# Autodesk Inventor assembly: mill_assembly
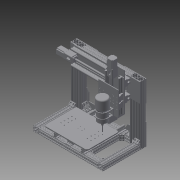
[picture p0: Inventor's stored thumbnail of the model, 180x180]
Saved by Autodesk Inventor 2014 (Build 180170000, 170)
## iProperties
Created: 2014-08-08
Part Number: mill_assembly
Document SubType Name: Assembly
Designer: Matthew
Author: Matthew
## Documents named in this file (45)
- C:\Users\Matthew\Documents\GitHub\CNC Mill\mill_assembly.iam
- C:\Users\Matthew\Documents\GitHub\CNC Mill\8020\2020.ipt
- C:\Users\Matthew\Documents\GitHub\CNC Mill\8020\2020_18in.ipt
- C:\Users\Matthew\Documents\GitHub\CNC Mill\8020\gusset_4138.ipt
- C:\Users\Matthew\Documents\GitHub\CNC Mill\8020\gusset_4134.ipt
- C:\Users\Matthew\Documents\GitHub\CNC Mill\mic6_plate.ipt
- C:\Users\Matthew\Documents\GitHub\CNC Mill\1605\1605_400mm.ipt
- C:\Users\Matthew\Documents\GitHub\CNC Mill\1605\1605_ballnut.ipt
- C:\Users\Matthew\Documents\GitHub\CNC Mill\nema23_motor_mount.ipt
- C:\Users\Matthew\Documents\GitHub\CNC Mill\6.35x10mm_coupler.ipt
- C:\Users\Matthew\Documents\GitHub\CNC Mill\sbr\sbr20\sbr20_400mm.ipt
- C:\Users\Matthew\Documents\GitHub\CNC Mill\HD16.ipt
- C:\Users\Matthew\Documents\GitHub\CNC Mill\nema23_HS8630.ipt
- C:\Users\Matthew\Documents\GitHub\CNC Mill\z-axis_mount_plate.ipt
- C:\Users\Matthew\Documents\GitHub\CNC Mill\y-axis_mount_plate.ipt
- C:\Users\Matthew\Documents\GitHub\CNC Mill\router_plate.ipt
- C:\Users\Matthew\Documents\GitHub\CNC Mill\router_mount.ipt
- C:\Users\Matthew\Documents\GitHub\CNC Mill\1617evs.ipt
- C:\Users\Matthew\Documents\GitHub\CNC Mill\ff12_mount.ipt
- C:\Users\Matthew\Documents\GitHub\CNC Mill\ff12.ipt
- C:\Users\Matthew\Documents\GitHub\CNC Mill\sbr\sbr20\sbr20_500mm.ipt
- C:\Users\Matthew\Documents\GitHub\CNC Mill\1605\1605_500mm.ipt
- C:\Users\Matthew\Documents\GitHub\CNC Mill\sbr\sbr20\sbr20_300mm.ipt
- C:\Users\Matthew\Documents\GitHub\CNC Mill\8020\2040_top_bar.ipt
- C:\Users\Matthew\Documents\GitHub\CNC Mill\8020\2040_uprights.ipt
- C:\Users\Matthew\Downloads\Imported Components\endmill 2 flute_finishing\endmill 2 flute_finishing.ipt
- C:\Users\Matthew\Downloads\Imported Components\User Library-ER COLLET\Assembly1.iam
- C:\Users\Matthew\Documents\GitHub\CNC Mill\8020\2020_rear.ipt
- C:\Users\Matthew\Documents\GitHub\CNC Mill\8020\2020_front.ipt
- C:\Users\Matthew\Documents\GitHub\CNC Mill\1605\1605_300mm.ipt
- C:\Users\Matthew\Documents\GitHub\CNC Mill\hd16_standoff.ipt
- C:\Users\Matthew\Documents\GitHub\CNC Mill\sbr20uu_standoff.ipt
- C:\Users\Matthew\Documents\GitHub\CNC Mill\versaframe\versaframe_30in.ipt
- C:\Users\Matthew\Documents\GitHub\CNC Mill\versaframe\versaframe_35in.ipt
- C:\Users\Matthew\Documents\GitHub\CNC Mill\versaframe\versaframe_7.5n.ipt
- C:\Users\Matthew\Documents\GitHub\CNC Mill\8020\2040-2040_left.iam
- C:\Users\Matthew\Documents\GitHub\CNC Mill\8020\2040-2040_right.iam
- C:\Users\Matthew\Documents\GitHub\CNC Mill\8020\2020-2040_right.iam
- C:\Users\Matthew\Documents\GitHub\CNC Mill\8020\2020-2040_left.iam
- C:\Users\Matthew\Documents\GitHub\CNC Mill\fk12.ipt
- C:\Users\Matthew\Documents\GitHub\CNC Mill\sbr\sbr20\sbr20uu.ipt
- C:\Users\Matthew\Documents\GitHub\CNC Mill\m6x1.ipt
- C:\Users\Matthew\Documents\GitHub\CNC Mill\m5x0.8.ipt
- C:\Users\Matthew\Documents\GitHub\CNC Mill\8020\SHCS bolt.ipt
- C:\Users\Matthew\Documents\GitHub\CNC Mill\8020\0.5in_tnut.iam
## Components (155 placed, 44 different names)
1. 2020_18in:1 — Mate:31, Mate:32, Mate:38, Mate:47, Mate:48, Flush:161, Flush:168, Mate:253
2. 2020_18in:2 — Mate:28, Mate:29, Mate:34, Mate:241, Flush:163, Mate:242, Flush:164, Mate:255, Flush:171, Flush:172, Mate:394
3. gusset_4138:1 — Mate:260, Mate:261, Flush:175
4. gusset_4138:2 — Mate:258, Mate:259, Mate:262, Flush:175
5. gusset_4134:1 — Mate:28, Mate:29, Mate:275
6. gusset_4134:2 — Mate:31, Mate:32, Mate:276, Insert:58, Insert:60, Insert:61, Insert:62
7. gusset_4134:3 — Mate:34, Flush:61, Flush:147, Mate:278
8. gusset_4134:4 — Mate:38, Flush:62, Flush:153, Mate:279
9. gusset_4134:6 — Mate:47, Mate:48, Flush:61, Flush:62, Mate:269, Flush:401, Flush:402, Flush:403
10. mic6_plate:1 — Mate:293, Flush:352, Insert:17, Insert:18, Insert:19, Insert:20, Insert:21, Insert:22, Insert:23, Insert:24, Insert:25, Insert:26, Insert:27, Insert:28, Insert:29, Insert:30, Insert:31, Insert:32, Insert:33, Insert:34, Insert:35, Insert:36, Flush:395
11. 1605_400mm:1 — Mate:108, Insert:2, Insert:13, Insert:16
12. 1605_ballnut:1 — Mate:108, Mate:133, Mate:134, Flush:75
13. nema23_motor_mount:1 — Mate:136, Mate:254, Flush:192, Flush:193, Mate:317, Flush:329, Flush:330
14. nema23_motor_mount:2 — Mate:154, Flush:321, Flush:322, Mate:316, Flush:327, Flush:328, Mate:364, Flush:376
15. 1605_ballnut:6 — Mate:158, Flush:90, Mate:159, Mate:282
16. 6.35x10mm_coupler:1 — Insert:4, Insert:14
17. sbr20_400mm:1 — Flush:136, Mate:247, Flush:191, Mate:318
18. sbr20_400mm:2 — Flush:136, Mate:248, Flush:190, Mate:328
19. HD16:1 — Mate:133, Mate:134, Flush:75, Flush:194, Mate:283, Mate:284, Mate:326, Mate:329, Flush:352, Mate:339
20. nema23_HS8630:1 — Mate:136, Flush:192, Flush:193
21. 6.35x10mm_coupler:2 — Insert:2
22. z-axis_mount_plate:1 — Mate:361, Flush:370, Flush:371, Flush:372, Flush:373, Mate:362, Mate:363, Flush:375, Mate:364, Flush:376, Flush:390, Flush:392
23. nema23_HS8630:2 — Mate:154, Insert:4, Flush:321, Flush:322
24. HD16:6 — Mate:158, Flush:90, Mate:159, Mate:186, Flush:120, Flush:121, Mate:210, Mate:211, Mate:378, Mate:379, Flush:389, Flush:390
25. y-axis_mount_plate:1 — Mate:177, Mate:199, Mate:200, Flush:135, Mate:206, Flush:137, Flush:184, Mate:267, Flush:396
26. nema23_motor_mount:4 — Mate:177, Flush:137, Flush:323, Flush:324, Mate:315, Flush:325, Flush:326
27. 6.35x10mm_coupler:3
28. nema23_HS8630:3 — Flush:323, Flush:324
29. 1605_ballnut:7 — Mate:240
30. HD16:7 — Mate:203, Mate:205, Mate:348, Mate:351, Mate:352, Flush:364
31. router_plate:1 — Mate:186, Flush:120, Flush:121, Mate:187, Flush:122, Flush:123, Mate:381, Flush:391, Flush:392, Mate:383, Flush:393, Flush:394, Insert:37, Insert:38, Insert:39, Insert:40, Insert:41, Insert:42, Insert:43, Insert:44, Insert:45, Insert:46, Insert:47, Insert:48, Insert:49, Insert:50, Insert:51, Insert:52, Insert:53, Insert:54, Insert:55, Insert:56
32. router_mount:1 — Insert:7, Mate:187, Flush:122, Flush:123, Mate:383, Flush:393, Flush:394
33. 1617evs:1 — Insert:7
34. ff12_mount:1 — Insert:9, Mate:256, Flush:331
35. ff12:1 — Insert:9, Insert:13
36. sbr20_500mm:1 — Flush:133, Mate:200, Mate:203, Flush:135, Mate:346, Flush:371, Mate:382
37. sbr20_500mm:2 — Flush:133, Mate:199, Mate:205, Mate:347
38. 1605_500mm:1 — Insert:11, Mate:240, Insert:15
39. ff12:2 — Insert:11, Insert:12
40. ff12_mount:2 — Insert:12, Mate:206
41. sbr20_300mm:1 — Flush:138, Mate:210, Flush:372, Mate:363, Flush:374, Flush:375, Mate:371
42. sbr20_300mm:2 — Flush:138, Mate:211, Flush:373, Mate:362, Flush:374, Mate:377
43. 2020:1 — Mate:223, Mate:230, Mate:233, Mate:248, Mate:250, Flush:169, Flush:190, Mate:389
44. 2020:2 — Mate:222, Mate:224, Mate:226, Mate:247, Mate:251, Flush:170, Flush:191, Mate:391
45. gusset_4134:8 — Mate:222, Flush:147, Mate:277
46. gusset_4134:9 — Mate:223, Flush:149, Flush:150, Flush:151, Mate:280, Flush:401
47. gusset_4134:11 — Mate:224, Flush:149, Mate:268
48. gusset_4134:12 — Mate:230, Flush:151, Mate:390
49. gusset_4134:13 — Mate:226, Flush:150, Mate:281
50. gusset_4134:14 — Flush:153, Mate:233
51. 2040_top_bar:1 — Mate:257, Flush:173, Flush:174, Mate:258, Mate:261, Flush:184, Mate:267, Flush:313, Flush:315
52. 2040_uprights:1 — Flush:161, Mate:241, Flush:167, Mate:252, Flush:168, Mate:253, Mate:257, Flush:173, Flush:174, Mate:259, Mate:262, Mate:269, Mate:276, Mate:311, Flush:314, Mate:314, Flush:319, Flush:320, Flush:396, Flush:398, Mate:385, Flush:400
53. endmill 2 flute_finishing:1
54. Assembly1:1 [sub-assembly]
55. 2040_uprights:2 — Flush:163, Mate:242, Flush:164, Mate:249, Flush:165, Flush:166, Mate:260, Mate:275, Flush:208, Mate:312, Flush:316, Mate:313, Flush:317, Flush:318, Mate:339, Mate:386, Flush:399, Flush:404, Mate:393
56. 2020_rear:1 — Mate:249, Flush:165, Flush:166, Mate:250, Mate:251, Flush:167, Mate:252, Flush:169, Flush:170, Mate:254, Mate:268, Mate:280, Flush:221, Mate:384, Mate:387, Mate:388, Mate:392
57. 2020_front:1 — Mate:255, Flush:171, Flush:172, Mate:256, Mate:277, Mate:278, Mate:279, Mate:281, Flush:331, Mate:390
58. 1605_300mm:1 — Insert:14, Mate:282
59. hd16_standoff:1 — Flush:194, Mate:283, Mate:284, Mate:293
60. versaframe_30in:1 — Flush:200, Flush:201, Mate:294, Flush:202, Flush:203, Mate:295, Flush:205, Flush:206, Flush:228, Flush:230
61. versaframe_30in:2 — Flush:200, Flush:201, Flush:204, Flush:221
62. versaframe_35in:1 — Mate:294, Flush:202, Flush:203, Flush:204, Flush:208, Flush:213, Mate:303, Flush:229
63. versaframe_35in:2 — Mate:295, Flush:205, Flush:206, Mate:297, Flush:209, Flush:210, Mate:304, Flush:231
64. versaframe_30in:3 — Mate:297, Flush:209, Flush:210, Flush:211, Flush:212, Flush:232, Flush:233, Mate:305
65. versaframe_30in:4 — Flush:211, Flush:212, Flush:213, Flush:220, Flush:308, Flush:235, Flush:309
66. versaframe_7.5n:1 — Flush:308, Flush:235, Flush:309, Flush:310, Flush:311, Mate:307, Mate:308
67. versaframe_7.5n:2 — Flush:232, Flush:233, Mate:305, Mate:306, Flush:234, Mate:309, Mate:310, Flush:312
68. versaframe_30in:5 — Flush:220, Flush:222, Mate:306, Flush:234, Flush:310
69. versaframe_30in:6 — Flush:222, Flush:311, Mate:307, Mate:308
70. versaframe_7.5n:3 — Mate:303, Flush:228, Flush:229
71. versaframe_7.5n:4 — Mate:304, Flush:230, Flush:231
72. versaframe_30in:7
73. versaframe_30in:8 — Mate:309, Mate:310, Flush:312
74. 2040-2040_left:1 [sub-assembly] — Mate:311, Flush:313, Flush:314
75. 2040-2040_right:1 [sub-assembly] — Mate:312, Flush:315, Flush:316
76. 2020-2040_right:1 [sub-assembly] — Mate:313, Flush:317, Flush:318
77. 2020-2040_left:1 [sub-assembly] — Mate:314, Flush:319, Flush:320
78. fk12:1 — Insert:15, Mate:315, Flush:325, Flush:326, Mate:382
79. fk12:2 — Mate:316, Flush:327, Flush:328
80. fk12:3 — Mate:317, Flush:329, Flush:330, Insert:16
81. sbr20uu:1 — Flush:332, Mate:319, Flush:333, Mate:332, Flush:347, Mate:333
82. sbr20uu:2 — Mate:318, Flush:332, Mate:319, Flush:333, Mate:326, Mate:335, Flush:349, Mate:336, Flush:395
83. sbr20uu:3 — Flush:344, Mate:327, Flush:345, Mate:328, Mate:329, Flush:350, Mate:337, Mate:338
84. sbr20uu:13 — Flush:344, Mate:327, Flush:345, Mate:330, Flush:346, Mate:331
85. sbr20uu_standoff:4 — Mate:330, Flush:346, Mate:331
86. sbr20uu_standoff:5 — Mate:332, Flush:347, Mate:333
87. sbr20uu_standoff:6 — Mate:335, Flush:349, Mate:336, Flush:353
88. sbr20uu_standoff:7 — Flush:350, Mate:337, Mate:338, Flush:353
89. m6x1:1 — Insert:24
90. m6x1:2 — Insert:21
91. m6x1:3 — Insert:17
92. m6x1:4 — Insert:20
93. m6x1:5 — Insert:18
94. m6x1:6 — Insert:19
95. m6x1:7 — Insert:22
96. m6x1:8 — Insert:23
97. m6x1:9 — Insert:28
98. m6x1:10 — Insert:27
99. m6x1:11 — Insert:32
100. m6x1:12 — Insert:26
101. m6x1:13 — Insert:29
102. m6x1:14 — Insert:30
103. m6x1:15 — Insert:25
104. m6x1:16 — Insert:31
105. m5x0.8:1 — Insert:36
106. m5x0.8:2 — Insert:34
107. m5x0.8:3 — Insert:33
108. m5x0.8:4 — Insert:35
109. sbr20uu:14 — Mate:347, Flush:362, Mate:348, Mate:355, Flush:366, Mate:356, Flush:370
110. sbr20uu:15 — Mate:353, Mate:354, Flush:365
111. sbr20uu:18 — Mate:346, Flush:362, Mate:358, Mate:359, Flush:368
112. sbr20uu:19 — Mate:357, Flush:367, Mate:360
113. sbr20uu_standoff:8 — Mate:353, Mate:354, Flush:365, Flush:369
114. hd16_standoff:2 — Mate:351, Mate:352, Flush:364, Mate:361
115. sbr20uu_standoff:9 — Mate:355, Flush:366, Mate:356
116. sbr20uu_standoff:10 — Mate:358, Mate:359, Flush:368
117. sbr20uu_standoff:11 — Mate:357, Flush:367, Mate:360, Flush:369
118. sbr20uu:22 — Mate:371
119. sbr20uu:23 — Flush:387, Flush:391
120. sbr20uu_standoff:12
121. sbr20uu_standoff:13 — Flush:388
122. sbr20uu:24
123. sbr20uu:25 — Mate:377, Flush:387, Mate:380
124. sbr20uu_standoff:14
125. sbr20uu_standoff:15 — Flush:388
126. hd16_standoff:3 — Mate:378, Mate:379, Flush:389, Mate:380, Mate:381
127. m6x1:18 — Insert:48
128. m6x1:19 — Insert:40
129. m6x1:20 — Insert:42
130. m6x1:21 — Insert:50
131. m6x1:22 — Insert:51
132. m6x1:23 — Insert:47
133. m6x1:24 — Insert:52
134. m6x1:25 — Insert:39
135. m6x1:26 — Insert:41
136. m6x1:27 — Insert:49
137. m6x1:28 — Insert:38
138. m6x1:29 — Insert:44
139. m6x1:30 — Insert:43
140. m6x1:31 — Insert:46
141. m6x1:32 — Insert:37
142. m6x1:33 — Insert:45
143. m5x0.8:5 — Insert:53
144. m5x0.8:6 — Insert:54
145. m5x0.8:7 — Insert:55
146. m5x0.8:8 — Insert:56
147. gusset_4138:5 — Mate:384, Flush:398, Mate:385
148. gusset_4138:6 — Mate:386, Flush:399, Mate:387
149. gusset_4134:15 — Mate:388, Mate:389, Flush:400, Flush:402
150. gusset_4134:16 — Mate:391, Flush:403, Flush:404, Mate:392, Flush:405
151. gusset_4134:17 — Mate:393, Mate:394, Flush:405
152. SHCS bolt:2 — Insert:58
153. 0.5in_tnut:2 [sub-assembly] — Insert:60
154. 0.5in_tnut:3 [sub-assembly] — Insert:61
155. SHCS bolt:3 — Insert:62
## Relationships (344: Mate 148, Flush 141, Insert 55)
- Mate:28: 2020_18in:2 ↔ gusset_4134:1
- Mate:29: 2020_18in:2 ↔ gusset_4134:1
- Mate:31: 2020_18in:1 ↔ gusset_4134:2
- Mate:32: 2020_18in:1 ↔ gusset_4134:2
- Mate:34: 2020_18in:2 ↔ gusset_4134:3
- Mate:38: 2020_18in:1 ↔ gusset_4134:4
- Mate:47: 2020_18in:1 ↔ gusset_4134:6
- Mate:48: 2020_18in:1 ↔ gusset_4134:6
- Mate:108: 1605_400mm:1 ↔ 1605_ballnut:1
- Flush:61: gusset_4134:3 ↔ gusset_4134:6
- Flush:62: gusset_4134:4 ↔ gusset_4134:6
- Mate:133: 1605_ballnut:1 ↔ HD16:1
- Mate:134: 1605_ballnut:1 ↔ HD16:1
- Flush:75: 1605_ballnut:1 ↔ HD16:1
- Insert:2 (-12.5 mm): 1605_400mm:1 ↔ 6.35x10mm_coupler:2
- Mate:136: nema23_motor_mount:1 ↔ nema23_HS8630:1
- Mate:154: nema23_motor_mount:2 ↔ nema23_HS8630:2
- Insert:4 (-7 mm): 6.35x10mm_coupler:1 ↔ nema23_HS8630:2
- Mate:158: 1605_ballnut:6 ↔ HD16:6
- Flush:90: 1605_ballnut:6 ↔ HD16:6
- Mate:159: 1605_ballnut:6 ↔ HD16:6
- [Mate]: nema23_motor_mount:4 ↔ nema23_HS8630:3
- [Insert] (-7 mm): 6.35x10mm_coupler:3 ↔ nema23_HS8630:3
- [Mate]: 1605_ballnut:7 ↔ HD16:7
- [Flush]: 1605_ballnut:7 ↔ HD16:7
- [Mate]: 1605_ballnut:7 ↔ HD16:7
- Mate:177: y-axis_mount_plate:1 ↔ nema23_motor_mount:4
- Insert:7: router_mount:1 ↔ 1617evs:1
- Mate:186: HD16:6 ↔ router_plate:1
- Flush:120 (-96.7994 mm): HD16:6 ↔ router_plate:1
- Flush:121 (64.897 mm): HD16:6 ↔ router_plate:1
- Mate:187: router_plate:1 ↔ router_mount:1
- Flush:122: router_plate:1 ↔ router_mount:1
- Flush:123 (44.45 mm): router_plate:1 ↔ router_mount:1
- Insert:9: ff12_mount:1 ↔ ff12:1
- Flush:133: sbr20_500mm:1 ↔ sbr20_500mm:2
- Mate:199: y-axis_mount_plate:1 ↔ sbr20_500mm:2
- Mate:200: y-axis_mount_plate:1 ↔ sbr20_500mm:1
- Mate:203 (19.9 mm): HD16:7 ↔ sbr20_500mm:1
- Mate:205 (19.9 mm): HD16:7 ↔ sbr20_500mm:2
- Flush:135: y-axis_mount_plate:1 ↔ sbr20_500mm:1
- Flush:136: sbr20_400mm:1 ↔ sbr20_400mm:2
- Insert:11: 1605_500mm:1 ↔ ff12:2
- Insert:12: ff12:2 ↔ ff12_mount:2
- Mate:206: y-axis_mount_plate:1 ↔ ff12_mount:2
- Insert:13: 1605_400mm:1 ↔ ff12:1
- Flush:137: y-axis_mount_plate:1 ↔ nema23_motor_mount:4
- Flush:138: sbr20_300mm:1 ↔ sbr20_300mm:2
- Mate:210 (11 mm): HD16:6 ↔ sbr20_300mm:1
- Mate:211 (11 mm): HD16:6 ↔ sbr20_300mm:2
- Mate:222: 2020:2 ↔ gusset_4134:8
- Flush:147: gusset_4134:3 ↔ gusset_4134:8
- Mate:223: 2020:1 ↔ gusset_4134:9
- Mate:224: 2020:2 ↔ gusset_4134:11
- Mate:226: 2020:2 ↔ gusset_4134:13
- Flush:149: gusset_4134:9 ↔ gusset_4134:11
- Mate:230: 2020:1 ↔ gusset_4134:12
- Flush:150: gusset_4134:9 ↔ gusset_4134:13
- Flush:151: gusset_4134:9 ↔ gusset_4134:12
- Flush:153: gusset_4134:4 ↔ gusset_4134:14
- Mate:233: 2020:1 ↔ gusset_4134:14
- Mate:240: 1605_ballnut:7 ↔ 1605_500mm:1
- Flush:161: 2020_18in:1 ↔ 2040_uprights:1
- Mate:241: 2020_18in:2 ↔ 2040_uprights:1
- Flush:163: 2020_18in:2 ↔ 2040_uprights:2
- Mate:242: 2020_18in:2 ↔ 2040_uprights:2
- Flush:164: 2020_18in:2 ↔ 2040_uprights:2
- Mate:247: sbr20_400mm:1 ↔ 2020:2
- Mate:248: sbr20_400mm:2 ↔ 2020:1
- Mate:249: 2040_uprights:2 ↔ 2020_rear:1
- Flush:165: 2040_uprights:2 ↔ 2020_rear:1
- Flush:166: 2040_uprights:2 ↔ 2020_rear:1
- Mate:250: 2020:1 ↔ 2020_rear:1
- Mate:251: 2020:2 ↔ 2020_rear:1
- Flush:167: 2040_uprights:1 ↔ 2020_rear:1
- Mate:252: 2040_uprights:1 ↔ 2020_rear:1
- Flush:168: 2020_18in:1 ↔ 2040_uprights:1
- Mate:253: 2020_18in:1 ↔ 2040_uprights:1
- Flush:169: 2020:1 ↔ 2020_rear:1
- Flush:170: 2020:2 ↔ 2020_rear:1
- Mate:254: nema23_motor_mount:1 ↔ 2020_rear:1
- Mate:255: 2020_18in:2 ↔ 2020_front:1
- Flush:171: 2020_18in:2 ↔ 2020_front:1
- Flush:172: 2020_18in:2 ↔ 2020_front:1
- Mate:256: ff12_mount:1 ↔ 2020_front:1
- Mate:257: 2040_top_bar:1 ↔ 2040_uprights:1
- Flush:173: 2040_top_bar:1 ↔ 2040_uprights:1
- Flush:174: 2040_top_bar:1 ↔ 2040_uprights:1
- Mate:258: gusset_4138:2 ↔ 2040_top_bar:1
- Mate:259: gusset_4138:2 ↔ 2040_uprights:1
- Mate:260: gusset_4138:1 ↔ 2040_uprights:2
- Mate:261: gusset_4138:1 ↔ 2040_top_bar:1
- Mate:262: gusset_4138:2 ↔ 2040_uprights:1
- Flush:175: gusset_4138:1 ↔ gusset_4138:2
- Flush:184: y-axis_mount_plate:1 ↔ 2040_top_bar:1
- Mate:267: y-axis_mount_plate:1 ↔ 2040_top_bar:1
- Mate:268: gusset_4134:11 ↔ 2020_rear:1
- Mate:269: gusset_4134:6 ↔ 2040_uprights:1
- Flush:190: sbr20_400mm:2 ↔ 2020:1
- Flush:191: sbr20_400mm:1 ↔ 2020:2
- Mate:275: gusset_4134:1 ↔ 2040_uprights:2
- Mate:276: gusset_4134:2 ↔ 2040_uprights:1
- Mate:277: gusset_4134:8 ↔ 2020_front:1
- Mate:278: gusset_4134:3 ↔ 2020_front:1
- Mate:279: gusset_4134:4 ↔ 2020_front:1
- Mate:280: gusset_4134:9 ↔ 2020_rear:1
- Mate:281: gusset_4134:13 ↔ 2020_front:1
- Insert:14 (-12.5 mm): 6.35x10mm_coupler:1 ↔ 1605_300mm:1
- Mate:282: 1605_ballnut:6 ↔ 1605_300mm:1
- Flush:192 (-0.889 mm): nema23_motor_mount:1 ↔ nema23_HS8630:1
- Flush:193: nema23_motor_mount:1 ↔ nema23_HS8630:1
- Flush:194: HD16:1 ↔ hd16_standoff:1
- Mate:283: HD16:1 ↔ hd16_standoff:1
- Mate:284: HD16:1 ↔ hd16_standoff:1
- Mate:293: mic6_plate:1 ↔ hd16_standoff:1
- Flush:200: versaframe_30in:1 ↔ versaframe_30in:2
- Flush:201: versaframe_30in:1 ↔ versaframe_30in:2
- Mate:294: versaframe_30in:1 ↔ versaframe_35in:1
- Flush:202: versaframe_30in:1 ↔ versaframe_35in:1
- Flush:203: versaframe_30in:1 ↔ versaframe_35in:1
- Flush:204: versaframe_30in:2 ↔ versaframe_35in:1
- Mate:295: versaframe_30in:1 ↔ versaframe_35in:2
- Flush:205: versaframe_30in:1 ↔ versaframe_35in:2
- Flush:206: versaframe_30in:1 ↔ versaframe_35in:2
- Flush:208: 2040_uprights:2 ↔ versaframe_35in:1
- Mate:297: versaframe_35in:2 ↔ versaframe_30in:3
- Flush:209: versaframe_35in:2 ↔ versaframe_30in:3
- Flush:210: versaframe_35in:2 ↔ versaframe_30in:3
- Flush:211: versaframe_30in:3 ↔ versaframe_30in:4
- Flush:212: versaframe_30in:3 ↔ versaframe_30in:4
- Flush:213: versaframe_35in:1 ↔ versaframe_30in:4
- Flush:220: versaframe_30in:4 ↔ versaframe_30in:5
- Flush:221: 2020_rear:1 ↔ versaframe_30in:2
- Flush:222: versaframe_30in:5 ↔ versaframe_30in:6
- Mate:303: versaframe_35in:1 ↔ versaframe_7.5n:3
- Flush:228: versaframe_30in:1 ↔ versaframe_7.5n:3
- Flush:229: versaframe_35in:1 ↔ versaframe_7.5n:3
- Mate:304: versaframe_35in:2 ↔ versaframe_7.5n:4
- Flush:230: versaframe_30in:1 ↔ versaframe_7.5n:4
- Flush:231: versaframe_35in:2 ↔ versaframe_7.5n:4
- Flush:232: versaframe_30in:3 ↔ versaframe_7.5n:2
- Flush:233: versaframe_30in:3 ↔ versaframe_7.5n:2
- Mate:305: versaframe_30in:3 ↔ versaframe_7.5n:2
- Mate:306: versaframe_7.5n:2 ↔ versaframe_30in:5
- Flush:234: versaframe_7.5n:2 ↔ versaframe_30in:5
- Flush:308: versaframe_30in:4 ↔ versaframe_7.5n:1
- Flush:235: versaframe_30in:4 ↔ versaframe_7.5n:1
- Flush:309: versaframe_30in:4 ↔ versaframe_7.5n:1
- Flush:310: versaframe_7.5n:1 ↔ versaframe_30in:5
- Flush:311: versaframe_7.5n:1 ↔ versaframe_30in:6
- Mate:307: versaframe_7.5n:1 ↔ versaframe_30in:6
- Mate:308: versaframe_7.5n:1 ↔ versaframe_30in:6
- Mate:309: versaframe_7.5n:2 ↔ versaframe_30in:8
- Mate:310: versaframe_7.5n:2 ↔ versaframe_30in:8
- Flush:312: versaframe_7.5n:2 ↔ versaframe_30in:8
- Mate:311: 2040_uprights:1 ↔ 2040-2040_left:1
- Flush:313: 2040_top_bar:1 ↔ 2040-2040_left:1
- Flush:314: 2040_uprights:1 ↔ 2040-2040_left:1
- Mate:312: 2040_uprights:2 ↔ 2040-2040_right:1
- Flush:315: 2040_top_bar:1 ↔ 2040-2040_right:1
- Flush:316: 2040_uprights:2 ↔ 2040-2040_right:1
- Mate:313: 2040_uprights:2 ↔ 2020-2040_right:1
- Flush:317: 2040_uprights:2 ↔ 2020-2040_right:1
- Flush:318: 2040_uprights:2 ↔ 2020-2040_right:1
- Mate:314: 2040_uprights:1 ↔ 2020-2040_left:1
- Flush:319: 2040_uprights:1 ↔ 2020-2040_left:1
- Flush:320: 2040_uprights:1 ↔ 2020-2040_left:1
- Flush:321 (-0.889 mm): nema23_motor_mount:2 ↔ nema23_HS8630:2
- Flush:322 (0.889 mm): nema23_motor_mount:2 ↔ nema23_HS8630:2
- Flush:323 (-0.889 mm): nema23_motor_mount:4 ↔ nema23_HS8630:3
- Flush:324: nema23_motor_mount:4 ↔ nema23_HS8630:3
- Insert:15: 1605_500mm:1 ↔ fk12:1
- Mate:315: nema23_motor_mount:4 ↔ fk12:1
- Flush:325 (6.1305 mm): nema23_motor_mount:4 ↔ fk12:1
- Flush:326 (6.1305 mm): nema23_motor_mount:4 ↔ fk12:1
- Mate:316: nema23_motor_mount:2 ↔ fk12:2
- Flush:327 (-6.1305 mm): nema23_motor_mount:2 ↔ fk12:2
- Flush:328 (6.1305 mm): nema23_motor_mount:2 ↔ fk12:2
- Mate:317: nema23_motor_mount:1 ↔ fk12:3
- Flush:329 (6.1305 mm): nema23_motor_mount:1 ↔ fk12:3
- Flush:330 (6.1305 mm): nema23_motor_mount:1 ↔ fk12:3
- Insert:16: 1605_400mm:1 ↔ fk12:3
- Flush:331: ff12_mount:1 ↔ 2020_front:1
- Mate:318: sbr20_400mm:1 ↔ sbr20uu:2
- Flush:332: sbr20uu:1 ↔ sbr20uu:2
- Mate:319 (20 mm): sbr20uu:1 ↔ sbr20uu:2
- Flush:333: sbr20uu:1 ↔ sbr20uu:2
- Mate:326 (-7.5 mm): HD16:1 ↔ sbr20uu:2
- Flush:344: sbr20uu:3 ↔ sbr20uu:13
- Mate:327 (20 mm): sbr20uu:3 ↔ sbr20uu:13
- Flush:345: sbr20uu:3 ↔ sbr20uu:13
- Mate:328: sbr20_400mm:2 ↔ sbr20uu:3
- Mate:329 (-7.5 mm): HD16:1 ↔ sbr20uu:3
- Mate:330: sbr20uu:13 ↔ sbr20uu_standoff:4
- Flush:346: sbr20uu:13 ↔ sbr20uu_standoff:4
- Mate:331: sbr20uu:13 ↔ sbr20uu_standoff:4
- Mate:332: sbr20uu:1 ↔ sbr20uu_standoff:5
- Flush:347: sbr20uu:1 ↔ sbr20uu_standoff:5
- Mate:333: sbr20uu:1 ↔ sbr20uu_standoff:5
- Mate:335: sbr20uu:2 ↔ sbr20uu_standoff:6
- Flush:349: sbr20uu:2 ↔ sbr20uu_standoff:6
- Mate:336: sbr20uu:2 ↔ sbr20uu_standoff:6
- Flush:350: sbr20uu:3 ↔ sbr20uu_standoff:7
- Mate:337: sbr20uu:3 ↔ sbr20uu_standoff:7
- Mate:338: sbr20uu:3 ↔ sbr20uu_standoff:7
- Flush:352 (-179.2 mm): mic6_plate:1 ↔ HD16:1
- Flush:353: sbr20uu_standoff:6 ↔ sbr20uu_standoff:7
- Mate:339 (201.2745 mm): HD16:1 ↔ 2040_uprights:2
- Insert:17: mic6_plate:1 ↔ m6x1:3
- Insert:18: mic6_plate:1 ↔ m6x1:5
- Insert:19: mic6_plate:1 ↔ m6x1:6
- Insert:20: mic6_plate:1 ↔ m6x1:4
- Insert:21: mic6_plate:1 ↔ m6x1:2
- Insert:22: mic6_plate:1 ↔ m6x1:7
- Insert:23: mic6_plate:1 ↔ m6x1:8
- Insert:24: mic6_plate:1 ↔ m6x1:1
- Insert:25: mic6_plate:1 ↔ m6x1:15
- Insert:26: mic6_plate:1 ↔ m6x1:12
- Insert:27: mic6_plate:1 ↔ m6x1:10
- Insert:28: mic6_plate:1 ↔ m6x1:9
- Insert:29: mic6_plate:1 ↔ m6x1:13
- Insert:30: mic6_plate:1 ↔ m6x1:14
- Insert:31: mic6_plate:1 ↔ m6x1:16
- Insert:32: mic6_plate:1 ↔ m6x1:11
- Insert:33: mic6_plate:1 ↔ m5x0.8:3
- Insert:34: mic6_plate:1 ↔ m5x0.8:2
- Insert:35: mic6_plate:1 ↔ m5x0.8:4
- Insert:36: mic6_plate:1 ↔ m5x0.8:1
- [Flush]: sbr20uu:14 ↔ sbr20uu:15
- [Mate] (60 mm): sbr20uu:14 ↔ sbr20uu:15
- [Flush]: sbr20uu:14 ↔ sbr20uu:15
- [Flush]: sbr20uu:18 ↔ sbr20uu:19
- [Mate] (70 mm): sbr20uu:18 ↔ sbr20uu:19
- [Flush]: sbr20uu:18 ↔ sbr20uu:19
- Mate:346: sbr20_500mm:1 ↔ sbr20uu:18
- Mate:347: sbr20_500mm:2 ↔ sbr20uu:14
- Flush:362: sbr20uu:14 ↔ sbr20uu:18
- Mate:348 (12.5 mm): HD16:7 ↔ sbr20uu:14
- Mate:351: HD16:7 ↔ hd16_standoff:2
- Mate:352: HD16:7 ↔ hd16_standoff:2
- Flush:364: HD16:7 ↔ hd16_standoff:2
- Mate:353: sbr20uu:15 ↔ sbr20uu_standoff:8
- Mate:354: sbr20uu:15 ↔ sbr20uu_standoff:8
- Flush:365: sbr20uu:15 ↔ sbr20uu_standoff:8
- Mate:355: sbr20uu:14 ↔ sbr20uu_standoff:9
- Flush:366: sbr20uu:14 ↔ sbr20uu_standoff:9
- Mate:356: sbr20uu:14 ↔ sbr20uu_standoff:9
- Mate:357: sbr20uu:19 ↔ sbr20uu_standoff:11
- Flush:367: sbr20uu:19 ↔ sbr20uu_standoff:11
- Mate:358: sbr20uu:18 ↔ sbr20uu_standoff:10
- Mate:359: sbr20uu:18 ↔ sbr20uu_standoff:10
- Flush:368: sbr20uu:18 ↔ sbr20uu_standoff:10
- Mate:360: sbr20uu:19 ↔ sbr20uu_standoff:11
- Flush:369: sbr20uu_standoff:8 ↔ sbr20uu_standoff:11
- Mate:361: z-axis_mount_plate:1 ↔ hd16_standoff:2
- Flush:370: z-axis_mount_plate:1 ↔ sbr20uu:14
- Flush:371 (-91.0209 mm): z-axis_mount_plate:1 ↔ sbr20_500mm:1
- Flush:372: z-axis_mount_plate:1 ↔ sbr20_300mm:1
- Flush:373: z-axis_mount_plate:1 ↔ sbr20_300mm:2
- Mate:362: z-axis_mount_plate:1 ↔ sbr20_300mm:2
- Mate:363: z-axis_mount_plate:1 ↔ sbr20_300mm:1
- Flush:374: sbr20_300mm:1 ↔ sbr20_300mm:2
- Flush:375: z-axis_mount_plate:1 ↔ sbr20_300mm:1
- Mate:364: nema23_motor_mount:2 ↔ z-axis_mount_plate:1
- Flush:376: nema23_motor_mount:2 ↔ z-axis_mount_plate:1
- [Flush]: sbr20uu:22 ↔ sbr20uu:23
- [Mate] (10 mm): sbr20uu:22 ↔ sbr20uu:23
- [Flush]: sbr20uu:22 ↔ sbr20uu:23
- [Mate]: sbr20uu:23 ↔ sbr20uu_standoff:13
- [Flush]: sbr20uu:23 ↔ sbr20uu_standoff:13
- [Mate]: sbr20uu:22 ↔ sbr20uu_standoff:12
- [Mate]: sbr20uu:22 ↔ sbr20uu_standoff:12
- [Flush]: sbr20uu:22 ↔ sbr20uu_standoff:12
- [Mate]: sbr20uu:23 ↔ sbr20uu_standoff:13
- Mate:371: sbr20_300mm:1 ↔ sbr20uu:22
- [Flush]: sbr20uu:24 ↔ sbr20uu:25
- [Mate] (10 mm): sbr20uu:24 ↔ sbr20uu:25
- [Flush]: sbr20uu:24 ↔ sbr20uu:25
- [Mate]: sbr20uu:25 ↔ sbr20uu_standoff:15
- [Flush]: sbr20uu:25 ↔ sbr20uu_standoff:15
- [Mate]: sbr20uu:24 ↔ sbr20uu_standoff:14
- [Mate]: sbr20uu:24 ↔ sbr20uu_standoff:14
- [Flush]: sbr20uu:24 ↔ sbr20uu_standoff:14
- [Mate]: sbr20uu:25 ↔ sbr20uu_standoff:15
- Mate:377: sbr20_300mm:2 ↔ sbr20uu:25
- Flush:387: sbr20uu:23 ↔ sbr20uu:25
- Flush:388: sbr20uu_standoff:13 ↔ sbr20uu_standoff:15
- Mate:378: HD16:6 ↔ hd16_standoff:3
- Mate:379: HD16:6 ↔ hd16_standoff:3
- Flush:389: HD16:6 ↔ hd16_standoff:3
- Mate:380 (-12.5 mm): sbr20uu:25 ↔ hd16_standoff:3
- Flush:390 (61 mm): z-axis_mount_plate:1 ↔ HD16:6
- Mate:381: router_plate:1 ↔ hd16_standoff:3
- Flush:391 (-59.3 mm): router_plate:1 ↔ sbr20uu:23
- Flush:392 (-8.9 mm): z-axis_mount_plate:1 ↔ router_plate:1
- Mate:382 (-40 mm): sbr20_500mm:1 ↔ fk12:1
- Mate:383: router_plate:1 ↔ router_mount:1
- Flush:393 (43.1 mm): router_plate:1 ↔ router_mount:1
- Flush:394: router_plate:1 ↔ router_mount:1
- Insert:37: router_plate:1 ↔ m6x1:32
- Insert:38: router_plate:1 ↔ m6x1:28
- Insert:39: router_plate:1 ↔ m6x1:25
- Insert:40: router_plate:1 ↔ m6x1:19
- Insert:41: router_plate:1 ↔ m6x1:26
- Insert:42: router_plate:1 ↔ m6x1:20
- Insert:43: router_plate:1 ↔ m6x1:30
- Insert:44: router_plate:1 ↔ m6x1:29
- Insert:45: router_plate:1 ↔ m6x1:33
- Insert:46: router_plate:1 ↔ m6x1:31
- Insert:47: router_plate:1 ↔ m6x1:23
- Insert:48: router_plate:1 ↔ m6x1:18
- Insert:49: router_plate:1 ↔ m6x1:27
- Insert:50: router_plate:1 ↔ m6x1:21
- Insert:51: router_plate:1 ↔ m6x1:22
- Insert:52: router_plate:1 ↔ m6x1:24
- Insert:53: router_plate:1 ↔ m5x0.8:5
- Insert:54: router_plate:1 ↔ m5x0.8:6
- Insert:55: router_plate:1 ↔ m5x0.8:7
- Insert:56: router_plate:1 ↔ m5x0.8:8
- Flush:395 (-92.4 mm): mic6_plate:1 ↔ sbr20uu:2
- Flush:396: y-axis_mount_plate:1 ↔ 2040_uprights:1
- Mate:384: 2020_rear:1 ↔ gusset_4138:5
- Flush:398: 2040_uprights:1 ↔ gusset_4138:5
- Mate:385: 2040_uprights:1 ↔ gusset_4138:5
- Mate:386: 2040_uprights:2 ↔ gusset_4138:6
- Flush:399: 2040_uprights:2 ↔ gusset_4138:6
- Mate:387: 2020_rear:1 ↔ gusset_4138:6
- Mate:388: 2020_rear:1 ↔ gusset_4134:15
- Mate:389: 2020:1 ↔ gusset_4134:15
- Flush:400 (-76.2 mm): 2040_uprights:1 ↔ gusset_4134:15
- Mate:390: gusset_4134:12 ↔ 2020_front:1
- Flush:401: gusset_4134:6 ↔ gusset_4134:9
- Flush:402: gusset_4134:6 ↔ gusset_4134:15
- Mate:391: 2020:2 ↔ gusset_4134:16
- Flush:403: gusset_4134:6 ↔ gusset_4134:16
- Flush:404 (-76.2 mm): 2040_uprights:2 ↔ gusset_4134:16
- Mate:392: 2020_rear:1 ↔ gusset_4134:16
- Mate:393: 2040_uprights:2 ↔ gusset_4134:17
- Mate:394: 2020_18in:2 ↔ gusset_4134:17
- Flush:405: gusset_4134:16 ↔ gusset_4134:17
- Insert:58: gusset_4134:2 ↔ SHCS bolt:2
- Insert:60: gusset_4134:2 ↔ 0.5in_tnut:2
- Insert:61: gusset_4134:2 ↔ 0.5in_tnut:3
- Insert:62: gusset_4134:2 ↔ SHCS bolt:3
## Named parameters: d373_d340 = -7 mm, d376_d338 = 0 mm, d379_d346 = 0 mm, d380_d347 = 0 mm, d381_d348 = 0 mm, yaxissbrspacing = 19.9 mm, zaxismount = 359.8418 mm, motoroffset = -0.889 mm, fk12offset = 6.1305 mm, d865_d806_d803_d800 = 0 mm, d866_d807_d804_d801 = 60 mm, d867_d808_d805_d802 = 0 mm, d876_d865_d806_d803_d800 = 0 mm, d877_d866_d807_d804_d801 = 70 mm, d878_d867_d808_d805_d802 = 0 mm, d918_d895 = 0 mm, d919_d876_d865_d806_d803_d800 = 0 mm, d920_d877_d866_d807_d804_d801 = 10 mm, d921_d878_d867_d808_d805_d802 = 0 mm, d922_d896 = 0 mm, d923_d897 = 0 mm, d924_d898 = 0 mm, d925_d899 = 0 mm, d926_d900 = 0 mm, d928_d918_d895 = 0 mm, d929_d919_d876_d865_d806_d803_d800 = 0 mm, d930_d920_d877_d866_d807_d804_d801 = 10 mm, d931_d921_d878_d867_d808_d805_d802 = 0 mm, d932_d922_d896 = 0 mm, d933_d923_d897 = 0 mm, d934_d924_d898 = 0 mm, d935_d925_d899 = 0 mm, d936_d926_d900 = 0 mm
